# Autodesk Inventor assembly: main
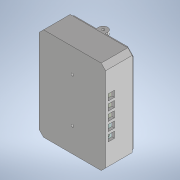
[picture p0: Inventor's stored thumbnail of the model, 180x180]
Saved by Autodesk Inventor 2020 (Build 240168000, 168)
## iProperties
Created: 2020-10-31
Part Number: main
Document SubType Name: Assembly
Designer: Leon
Author: Leon
## Documents named in this file (4)
- C:\Users\Leon\Google Drive\FAKS\ZAVRSNI\Inventor\03-assems\main.iam
- C:\Users\Leon\Google Drive\FAKS\ZAVRSNI\Inventor\01-sub_assems\AmpLogger.ipt
- C:\Users\Leon\Google Drive\FAKS\ZAVRSNI\Inventor\00-parts\Casing-v2.ipt
- C:\Users\Leon\Google Drive\FAKS\ZAVRSNI\Inventor\00-parts\Casing-v2-top.ipt
## Components (3 placed, 3 different names)
1. AmpLogger:1 — Mate:1, Mate:2, Flush:1
2. Casing-v2:1 — Rigid:2, Mate:1, Mate:2, Flush:1
3. Casing-v2-top:1 — Rigid:2
## Relationships (4: Mate 2, WeldJoint 1, Flush 1)
- Rigid:2 [WeldJoint]: Casing-v2:1 ↔ Casing-v2-top:1
- Mate:1 (7 mm): AmpLogger:1 ↔ Casing-v2:1
- Mate:2 (10 mm): AmpLogger:1 ↔ Casing-v2:1
- Flush:1: AmpLogger:1 ↔ Casing-v2:1
